# Autodesk Inventor assembly: mx106-contre-axe
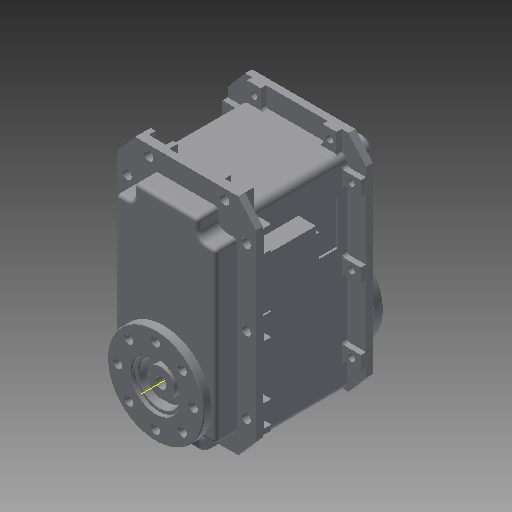
[picture p0: Inventor's stored thumbnail of the model, 512x512]
Saved by Autodesk Inventor 2018 (Build 220112000, 112)
## iProperties
Created: 2018-05-02
Part Number: mx106-contre-axe
Document SubType Name: Assembly
Designer: medrimonia
Author: medrimonia
## Documents named in this file (3)
- C:\Users\medrimonia\Dropbox\SigmaBan\SigmaBanV2.1\dynamixel\motors\mx106-contre-axe.iam
- C:\Users\medrimonia\Dropbox\SigmaBan\SigmaBanV2.1\MX-106T.ipt
- C:\Users\medrimonia\Dropbox\SigmaBan\SigmaBanV2.1\dynamixel\horn\HN05-i101.ipt
## Components (2 placed, 2 different names)
1. MX-106T:1 — Mate:1, Flush:1
2. HN05-i101:1 — Mate:1, Flush:1
## Relationships (2: Mate 1, Flush 1)
- Mate:1: MX-106T:1 ↔ HN05-i101:1
- Flush:1 (3 mm): MX-106T:1 ↔ HN05-i101:1
